# Autodesk Inventor assembly: WCP SS
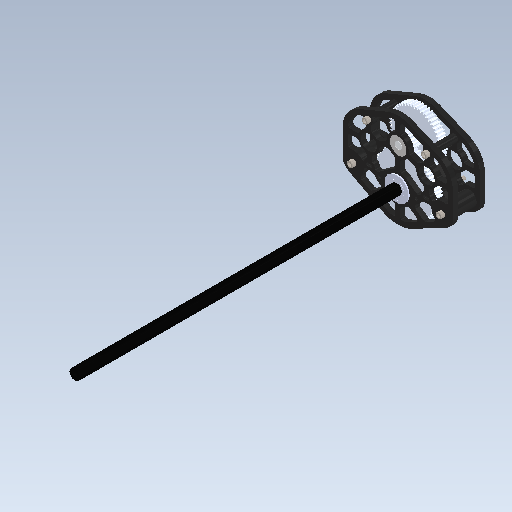
[picture p0: Inventor's stored thumbnail of the model, 512x512]
Saved by Autodesk Inventor 2021.1 (Build 251245000, 245)
## iProperties
Created: 2013-12-10
Part Number: WCP SS
Description: STEP AP214
Document SubType Name: Assembly
Designer: aidan
Sending System: SolidWorks 2013
Preprocessor: SwSTEP 2.0
Title: 217-3421-STEP.STEP
Revision Number: ANY
## Documents named in this file (16)
- C:\Users\Spade\OneDrive\Documents\t3-cad\CAD\WCP SS.iam
- C:\Users\Spade\OneDrive\Documents\t3-cad\CAD\Generic and Stock\217-2733.ipt
- C:\Users\Spade\OneDrive\Documents\t3-cad\CAD\Generic and Stock\217-3100-001_14t.ipt
- C:\Users\Spade\OneDrive\Documents\t3-cad\CAD\Generic and Stock\217-2711-002 Rev1_50t.ipt
- C:\Users\Spade\OneDrive\Documents\t3-cad\CAD\Generic and Stock\217-2714-002 Rev1_60t.ipt
- C:\Users\Spade\OneDrive\Documents\t3-cad\CAD\Generic and Stock\217-3421-003 Rev1.ipt
- C:\Users\Spade\OneDrive\Documents\t3-cad\CAD\Generic and Stock\217-3421-005 Rev1.ipt
- C:\Users\Spade\OneDrive\Documents\t3-cad\CAD\Generic and Stock\217-3421-006 Rev1.ipt
- C:\Users\Spade\OneDrive\Documents\t3-cad\CAD\Generic and Stock\217-3261-001 Rev1.ipt
- C:\Users\Spade\OneDrive\Documents\t3-cad\CAD\Generic and Stock\217-3421-007 Rev1.ipt
- C:\Users\Spade\OneDrive\Documents\t3-cad\CAD\Generic and Stock\217-3421-008 Rev1.ipt
- C:\Users\Spade\OneDrive\Documents\t3-cad\CAD\Generic and Stock\217-3421-009 Rev1.ipt
- C:\Users\Spade\OneDrive\Documents\t3-cad\CAD\Generic and Stock\217-3421-010 Rev1.ipt
- C:\Users\Spade\OneDrive\Documents\t3-cad\CAD\16in THUNDERSHAFT.ipt
- C:\Users\Spade\OneDrive\Documents\t3-cad\CAD\Generic and Stock\217-2734.ipt
- C:\Users\Spade\OneDrive\Documents\t3-cad\CAD\WCS SS Plate.ipt
## Components (24 placed, 22 different names)
1. 217-2733_2 — Mate:14, Mate:15, Mate:16, Mate:17, Mate:21
2. 217-2733_3 — Mate:12, Mate:13
3. 217-3100-001_14t_8 — Flush:4, Flush:5, Mate:18, Mate:19, Mate:20, Flush:7, Rotation:1
4. 217-2711-002 Rev1_50t_9 — Flush:4, Flush:5, Mate:18, Mate:21
5. 217-2714-002 Rev1_60t_10 — Mate:22, Mate:23, Flush:7, Rotation:1, Mate:26
6. 217-3421-003 Rev1_16 — Mate:16, Mate:17, Mate:19, Mate:20
7. 217-3421-005 Rev1_18 — Flush:8, Mate:27, Mate:29
8. 217-3421-005 Rev1_19 — Flush:8, Mate:28, Mate:40
9. 217-3421-006 Rev1_20 — Flush:3, Mate:11, Mate:39
10. 217-3421-006 Rev1_21 — Mate:9, Mate:10, Flush:3, Mate:38
11. 217-3261-001 Rev1_22 — Mate:24, Mate:25, Mate:26
12. 217-3421-007 Rev1_23 — Flush:11, Mate:38
13. 217-3421-007 Rev1_24 — Flush:11, Mate:39, Mate:42
14. 217-3421-008 Rev1_25 — Mate:28, Flush:9, Mate:31, Mate:41
15. 217-3421-008 Rev1_26 — Mate:27, Flush:9, Mate:30
16. 217-3421-009 Rev1_30 — Flush:6, Mate:33, Mate:34
17. 217-3421-010 Rev1_31 — Flush:10, Mate:37
18. 217-3421-010 Rev1_32 — Flush:10, Mate:35, Mate:36
19. 16in THUNDERSHAFT:1 — Mate:1, Mate:2, Mate:3, Mate:4, Flush:1, Mate:22, Mate:23, Mate:24, Mate:25
20. 217-2734:1 — Mate:1, Mate:2, Mate:7, Mate:8
21. 217-2734:2 — Mate:3, Mate:4, Mate:5, Mate:6, Flush:1
22. WCS SS Plate:1 — Mate:5, Mate:6, Flush:2, Mate:10, Mate:11, Mate:14, Mate:15, Mate:29, Mate:30, Mate:31, Mate:32, Mate:33, Mate:34, Mate:35, Mate:36, Mate:37
23. WCS SS Plate:2 — Mate:7, Mate:8, Flush:2, Mate:9, Mate:12, Mate:13, Mate:40, Mate:41, Mate:42
24. 217-3421-009 Rev1:5 — Flush:6, Mate:32
## Relationships (54: Mate 42, Flush 11, RelateRotation 1)
- Mate:1: 16in THUNDERSHAFT:1 ↔ 217-2734:1
- Mate:2: 16in THUNDERSHAFT:1 ↔ 217-2734:1
- Mate:3: 16in THUNDERSHAFT:1 ↔ 217-2734:2
- Mate:4: 16in THUNDERSHAFT:1 ↔ 217-2734:2
- Mate:5: 217-2734:2 ↔ WCS SS Plate:1
- Mate:6: 217-2734:2 ↔ WCS SS Plate:1
- Flush:1: 16in THUNDERSHAFT:1 ↔ 217-2734:2
- Mate:7: 217-2734:1 ↔ WCS SS Plate:2
- Mate:8: 217-2734:1 ↔ WCS SS Plate:2
- Flush:2: WCS SS Plate:1 ↔ WCS SS Plate:2
- Mate:9: 217-3421-006 Rev1_21 ↔ WCS SS Plate:2
- Mate:10: 217-3421-006 Rev1_21 ↔ WCS SS Plate:1
- Flush:3: 217-3421-006 Rev1_20 ↔ 217-3421-006 Rev1_21
- Mate:11: 217-3421-006 Rev1_20 ↔ WCS SS Plate:1
- Mate:12: 217-2733_3 ↔ WCS SS Plate:2
- Mate:13: 217-2733_3 ↔ WCS SS Plate:2
- Mate:14: 217-2733_2 ↔ WCS SS Plate:1
- Mate:15: 217-2733_2 ↔ WCS SS Plate:1
- Mate:16: 217-2733_2 ↔ 217-3421-003 Rev1_16
- Mate:17: 217-2733_2 ↔ 217-3421-003 Rev1_16
- Flush:4: 217-3100-001_14t_8 ↔ 217-2711-002 Rev1_50t_9
- Flush:5: 217-3100-001_14t_8 ↔ 217-2711-002 Rev1_50t_9
- Mate:18: 217-3100-001_14t_8 ↔ 217-2711-002 Rev1_50t_9
- Mate:19: 217-3100-001_14t_8 ↔ 217-3421-003 Rev1_16
- Mate:20: 217-3100-001_14t_8 ↔ 217-3421-003 Rev1_16
- Mate:21: 217-2733_2 ↔ 217-2711-002 Rev1_50t_9
- Flush:6: 217-3421-009 Rev1_30 ↔ 217-3421-009 Rev1:5
- Mate:22: 217-2714-002 Rev1_60t_10 ↔ 16in THUNDERSHAFT:1
- Mate:23: 217-2714-002 Rev1_60t_10 ↔ 16in THUNDERSHAFT:1
- Flush:7: 217-3100-001_14t_8 ↔ 217-2714-002 Rev1_60t_10
- Rotation:1 [RelateRotation] (1 ul): 217-3100-001_14t_8 ↔ 217-2714-002 Rev1_60t_10
- Mate:24: 217-3261-001 Rev1_22 ↔ 16in THUNDERSHAFT:1
- Mate:25: 217-3261-001 Rev1_22 ↔ 16in THUNDERSHAFT:1
- Mate:26: 217-2714-002 Rev1_60t_10 ↔ 217-3261-001 Rev1_22
- Flush:8: 217-3421-005 Rev1_18 ↔ 217-3421-005 Rev1_19
- Mate:27: 217-3421-005 Rev1_18 ↔ 217-3421-008 Rev1_26
- Mate:28: 217-3421-005 Rev1_19 ↔ 217-3421-008 Rev1_25
- Flush:9: 217-3421-008 Rev1_25 ↔ 217-3421-008 Rev1_26
- Mate:29: 217-3421-005 Rev1_18 ↔ WCS SS Plate:1
- Mate:30: 217-3421-008 Rev1_26 ↔ WCS SS Plate:1
- Mate:31: 217-3421-008 Rev1_25 ↔ WCS SS Plate:1
- Mate:32: WCS SS Plate:1 ↔ 217-3421-009 Rev1:5
- Mate:33: 217-3421-009 Rev1_30 ↔ WCS SS Plate:1
- Mate:34: 217-3421-009 Rev1_30 ↔ WCS SS Plate:1
- Flush:10: 217-3421-010 Rev1_31 ↔ 217-3421-010 Rev1_32
- Flush:11: 217-3421-007 Rev1_23 ↔ 217-3421-007 Rev1_24
- Mate:35: 217-3421-010 Rev1_32 ↔ WCS SS Plate:1
- Mate:36: 217-3421-010 Rev1_32 ↔ WCS SS Plate:1
- Mate:37: 217-3421-010 Rev1_31 ↔ WCS SS Plate:1
- Mate:38: 217-3421-006 Rev1_21 ↔ 217-3421-007 Rev1_23
- Mate:39: 217-3421-006 Rev1_20 ↔ 217-3421-007 Rev1_24
- Mate:40: 217-3421-005 Rev1_19 ↔ WCS SS Plate:2
- Mate:41: 217-3421-008 Rev1_25 ↔ WCS SS Plate:2
- Mate:42: 217-3421-007 Rev1_24 ↔ WCS SS Plate:2
